# Autodesk Inventor assembly: Intake
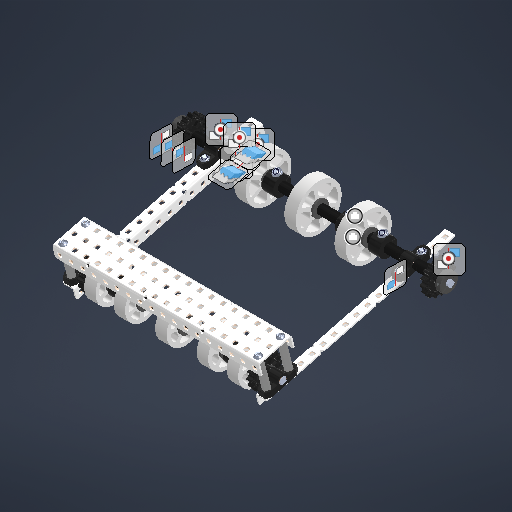
[picture p0: Inventor's stored thumbnail of the model, 512x512]
Saved by Autodesk Inventor 2025 (Build 290162000, 162)
## iProperties
Created: 2024-12-18
Part Number: Intake
Document SubType Name: Assembly
Designer: Juan
Author: Juan
## Documents named in this file (26)
- C:\Users\Juan\Documents\GitHub\ATUM-VRC-High-Stakes-CAD\Protobot\Intake.iam
- C:\Users\Juan\Documents\GitHub\ATUM-VRC-High-Stakes-CAD\VEX-CAD-Inventor\Motion\Shaft HS\Shaft HS\Shaft HS 9.0 in.ipt
- C:\Users\Juan\Documents\GitHub\ATUM-VRC-High-Stakes-CAD\VEX-CAD-Inventor\Motion\Shaft HS\Shaft HS.ipt
- C:\Users\Juan\Documents\GitHub\ATUM-VRC-High-Stakes-CAD\VEX-CAD-Inventor\Structure\Angle\Aluminum 1x1\Alu Angle 1x1x17.ipt
- C:\Users\Juan\Documents\GitHub\ATUM-VRC-High-Stakes-CAD\VEX-CAD-Inventor\Motion\Shaft HS\HS Pillow Bearing Block.ipt
- C:\Users\Juan\Documents\GitHub\ATUM-VRC-High-Stakes-CAD\VEX-CAD-Inventor\Motion\Sprockets\6P Sprocket\6P 16T Sprocket, No Insert.iam
- C:\Users\Juan\Documents\GitHub\ATUM-VRC-High-Stakes-CAD\VEX-CAD-Inventor\Motion\Sprockets\6P Sprocket.iam
- C:\Users\Juan\Documents\GitHub\ATUM-VRC-High-Stakes-CAD\VEX-CAD-Inventor\Structure\Hardware\Screw Steel - Star\SScrew Star Threaded .375.ipt
- C:\Users\Juan\Documents\GitHub\ATUM-VRC-High-Stakes-CAD\VEX-CAD-Inventor\Structure\Hardware\Screw Steel - Star.ipt
- C:\Users\Juan\Documents\GitHub\ATUM-VRC-High-Stakes-CAD\VEX-CAD-Inventor\Structure\C Channel\Aluminum 1x3x1\Alu C 1x3x1x18.ipt
- C:\Users\Juan\Documents\GitHub\ATUM-VRC-High-Stakes-CAD\VEX-CAD-Inventor\Structure\Standoff\Standoff 1.50.ipt
- C:\Users\Juan\Documents\GitHub\ATUM-VRC-High-Stakes-CAD\VEX-CAD-Inventor\Structure\Standoff.ipt
- C:\Users\Juan\Documents\GitHub\ATUM-VRC-High-Stakes-CAD\VEX-CAD-Inventor\Motion\1-Post Bearing Flat Hex Retainer.ipt
- C:\Users\Juan\Documents\GitHub\ATUM-VRC-High-Stakes-CAD\VEX-CAD-Inventor\Motion\Shaft HS\Shaft HS\Shaft HS 12.0 in.ipt
- C:\Users\Juan\Documents\GitHub\ATUM-VRC-High-Stakes-CAD\VEX-CAD-Inventor\Motion\Shaft HS\HS Shaft Collar.ipt
- C:\Users\Juan\Documents\GitHub\ATUM-VRC-High-Stakes-CAD\VEX-CAD-Inventor\Motion\Shaft HS\HS Spacer\HSpacer .5000.ipt
- C:\Users\Juan\Documents\GitHub\ATUM-VRC-High-Stakes-CAD\VEX-CAD-Inventor\Motion\Shaft HS\HS Spacer.ipt
- C:\Users\Juan\Documents\GitHub\ATUM-VRC-High-Stakes-CAD\VEX-CAD-Inventor\Motion\Shaft HS\Low Profile HS Shaft Collar.ipt
- C:\Users\Juan\Documents\GitHub\ATUM-VRC-High-Stakes-CAD\VEX-CAD-Inventor\Motion\Shaft HS\HS Spacer\HSpacer .2500.ipt
- C:\Users\Juan\Documents\GitHub\ATUM-VRC-High-Stakes-CAD\Protobot\2.0 Flex Wheel with Insert.iam
- C:\Users\Juan\Documents\GitHub\ATUM-VRC-High-Stakes-CAD\VEX-CAD-Inventor\Structure\Hardware\Nut Thin Nylock.ipt
- C:\Users\Juan\Documents\GitHub\ATUM-VRC-High-Stakes-CAD\VEX-CAD-Inventor\Structure\Hardware\Screw Steel - Star\SScrew Star Smooth .625.ipt
- C:\Users\Juan\Documents\GitHub\ATUM-VRC-High-Stakes-CAD\VEX-CAD-Inventor\Motion\Shaft HS\HS Spacer\HSpacer .1250.ipt
- C:\Users\Juan\Documents\GitHub\ATUM-VRC-High-Stakes-CAD\VEX-CAD-Inventor\Motion\Shaft HS\HS Spacer\HSpacer .0625.ipt
- C:\Users\Juan\Documents\GitHub\ATUM-VRC-High-Stakes-CAD\VEX-CAD-Inventor\Structure\Hardware\Screw Steel - Star\SScrew Star Smooth .375.ipt
- C:\Users\Juan\Documents\GitHub\ATUM-VRC-High-Stakes-CAD\Protobot\1.625 Flex Wheel with Insert.iam
## Components (88 placed, 20 different names)
1. Shaft HS 9.0 in:1
2. Alu Angle 1x1x17:1
3. HS Pillow Bearing Block:4
4. Alu Angle 1x1x17:2
5. HS Pillow Bearing Block:1
6. HS Pillow Bearing Block:2
7. 6P 16T Sprocket, No Insert:1 [sub-assembly]
8. 6P 16T Sprocket, No Insert:2 [sub-assembly]
9. SScrew Star Threaded .375:1
10. Alu C 1x3x1x18:1
11. Standoff 1.50:1
12. Standoff 1.50:2
13. Standoff 1.50:3
14. Standoff 1.50:4
15. 1-Post Bearing Flat Hex Retainer:1
16. HS Pillow Bearing Block:3
17. Shaft HS 12.0 in:2
18. 6P 16T Sprocket, No Insert:3 [sub-assembly]
19. 6P 16T Sprocket, No Insert:4 [sub-assembly]
20. HS Shaft Collar:1
21. HS Shaft Collar:2
22. HSpacer .5000:1
23. HSpacer .5000:2
24. HSpacer .5000:3
25. HSpacer .5000:4
26. Low Profile HS Shaft Collar:1
27. Low Profile HS Shaft Collar:2
28. HS Shaft Collar:3
29. HS Shaft Collar:4
30. HSpacer .2500:5
31. HSpacer .2500:6
32. 2.0 Flex Wheel with Insert:1 [sub-assembly]
33. 2.0 Flex Wheel with Insert:2 [sub-assembly]
34. 2.0 Flex Wheel with Insert:3 [sub-assembly]
35. HSpacer .5000:7
36. Nut Thin Nylock:1
37. HSpacer .5000:8
38. SScrew Star Smooth .625:2
39. SScrew Star Smooth .625:3
40. SScrew Star Smooth .625:4
41. SScrew Star Smooth .625:5
42. Nut Thin Nylock:2
43. Nut Thin Nylock:3
44. Nut Thin Nylock:4
45. HSpacer .5000:9
46. HSpacer .5000:10
47. HSpacer .1250:11
48. HSpacer .1250:12
49. HSpacer .0625:13
50. HSpacer .1250:14
51. HSpacer .1250:15
52. HSpacer .0625:16
53. HSpacer .0625:17
54. Nut Thin Nylock:5
55. Nut Thin Nylock:6
56. Nut Thin Nylock:7
57. Nut Thin Nylock:8
58. SScrew Star Smooth .375:6
59. SScrew Star Smooth .375:7
60. SScrew Star Smooth .375:8
61. SScrew Star Smooth .375:9
62. SScrew Star Smooth .375:10
63. SScrew Star Smooth .375:11
64. SScrew Star Smooth .375:12
65. SScrew Star Smooth .375:13
66. SScrew Star Smooth .375:14
67. SScrew Star Smooth .375:15
68. SScrew Star Smooth .375:16
69. SScrew Star Smooth .375:17
70. 1.625 Flex Wheel with Insert:1 [sub-assembly]
71. 1.625 Flex Wheel with Insert:2 [sub-assembly]
72. 1.625 Flex Wheel with Insert:3 [sub-assembly]
73. 1.625 Flex Wheel with Insert:4 [sub-assembly]
74. 1.625 Flex Wheel with Insert:5 [sub-assembly]
75. HSpacer .5000:18
76. HSpacer .1250:19
77. HSpacer .1250:20
78. HSpacer .5000:21
79. HSpacer .5000:22
80. HSpacer .5000:23
81. HS Shaft Collar:5
82. Nut Thin Nylock:9
83. SScrew Star Smooth .625:18
84. HS Shaft Collar:6
85. Nut Thin Nylock:10
86. SScrew Star Smooth .625:19
87. HSpacer .1250:24
88. HSpacer .1250:25
## Relationships (158: Mate 117, WeldJoint 30, CylindricalJoint 9, Flush 1, Angle 1)
- [Mate]: Alu Angle 1x1x17:1 ↔ HS Pillow Bearing Block:1
- [Mate]: Alu Angle 1x1x17:1 ↔ HS Pillow Bearing Block:1
- [Mate]: Alu Angle 1x1x17:1 ↔ HS Pillow Bearing Block:1
- [Mate]: Shaft HS 9.0 in:1 ↔ HS Pillow Bearing Block:1
- [Mate]: Alu Angle 1x1x17:2 ↔ HS Pillow Bearing Block:2
- [Mate]: Alu Angle 1x1x17:2 ↔ HS Pillow Bearing Block:2
- [Mate]: Alu Angle 1x1x17:2 ↔ HS Pillow Bearing Block:2
- [Mate]: Shaft HS 9.0 in:1 ↔ HS Pillow Bearing Block:2
- [Mate]: Shaft HS 9.0 in:1 ↔ 6P 16T Sprocket, No Insert:2
- [Mate]: Shaft HS 9.0 in:1 ↔ 6P 16T Sprocket, No Insert:1
- [Mate]: Alu Angle 1x1x17:1 ↔ SScrew Star Threaded .375:1
- [Mate]: Alu Angle 1x1x17:1 ↔ 6P 16T Sprocket, No Insert:2
- [Mate]: Alu Angle 1x1x17:1 ↔ SScrew Star Threaded .375:1
- [Mate]: Alu Angle 1x1x17:1 ↔ Alu Angle 1x1x17:2
- [Mate]: HS Pillow Bearing Block:1 ↔ Standoff 1.50:1
- [Mate]: HS Pillow Bearing Block:1 ↔ Standoff 1.50:2
- [Mate]: HS Pillow Bearing Block:1 ↔ Standoff 1.50:1
- [Mate]: HS Pillow Bearing Block:1 ↔ Standoff 1.50:2
- [Mate]: Alu C 1x3x1x18:1 ↔ Standoff 1.50:1
- [Mate]: Alu C 1x3x1x18:1 ↔ Standoff 1.50:2
- [Mate]: Alu C 1x3x1x18:1 ↔ Standoff 1.50:2
- [Mate]: HS Pillow Bearing Block:2 ↔ Standoff 1.50:4
- [Mate]: HS Pillow Bearing Block:2 ↔ Standoff 1.50:3
- [Mate]: HS Pillow Bearing Block:2 ↔ Standoff 1.50:4
- [Mate]: HS Pillow Bearing Block:2 ↔ Standoff 1.50:3
- [Mate]: Alu C 1x3x1x18:1 ↔ Standoff 1.50:3
- [Mate]: Alu Angle 1x1x17:2 ↔ HS Pillow Bearing Block:3
- [Mate]: Alu Angle 1x1x17:2 ↔ HS Pillow Bearing Block:3
- [Mate]: Alu Angle 1x1x17:2 ↔ HS Pillow Bearing Block:3
- [Mate]: Shaft HS 12.0 in:2 ↔ 6P 16T Sprocket, No Insert:3
- [Mate]: Shaft HS 12.0 in:2 ↔ 6P 16T Sprocket, No Insert:4
- [Mate]: Shaft HS 12.0 in:2 ↔ 2.0 Flex Wheel with Insert:3
- [Mate]: Shaft HS 12.0 in:2 ↔ 2.0 Flex Wheel with Insert:2
- [Mate]: Shaft HS 12.0 in:2 ↔ 2.0 Flex Wheel with Insert:1
- [Mate]: Shaft HS 12.0 in:2 ↔ HSpacer .5000:4
- [Mate]: Shaft HS 12.0 in:2 ↔ HSpacer .5000:4
- [Mate]: Shaft HS 12.0 in:2 ↔ HS Shaft Collar:1
- [Mate]: Shaft HS 12.0 in:2 ↔ HS Shaft Collar:1
- [Mate]: Shaft HS 12.0 in:2 ↔ HSpacer .5000:1
- [Mate]: Shaft HS 12.0 in:2 ↔ HSpacer .5000:1
- [Mate]: HSpacer .5000:1 ↔ HSpacer .5000:4
- [Mate]: HS Shaft Collar:1 ↔ HSpacer .5000:4
- [Mate]: HS Shaft Collar:1 ↔ 2.0 Flex Wheel with Insert:3
- [Mate]: HSpacer .5000:1 ↔ 2.0 Flex Wheel with Insert:2
- [Mate]: Shaft HS 12.0 in:2 ↔ HS Shaft Collar:2
- [Mate]: Shaft HS 12.0 in:2 ↔ HS Shaft Collar:2
- [Mate]: Shaft HS 12.0 in:2 ↔ HSpacer .5000:3
- [Mate]: Shaft HS 12.0 in:2 ↔ HSpacer .5000:3
- [Mate]: Shaft HS 12.0 in:2 ↔ HSpacer .5000:2
- [Mate]: Shaft HS 12.0 in:2 ↔ HSpacer .5000:2
- [Mate]: HSpacer .5000:2 ↔ 2.0 Flex Wheel with Insert:2
- [Mate]: HSpacer .5000:2 ↔ HSpacer .5000:3
- [Mate]: HS Shaft Collar:2 ↔ HSpacer .5000:3
- [Mate]: HS Shaft Collar:2 ↔ 2.0 Flex Wheel with Insert:1
- [Mate] (36.1696 mm): Alu Angle 1x1x17:1 ↔ 2.0 Flex Wheel with Insert:3
- [Mate]: Shaft HS 12.0 in:2 ↔ Low Profile HS Shaft Collar:2
- [Mate]: Shaft HS 12.0 in:2 ↔ Low Profile HS Shaft Collar:2
- [Mate]: 6P 16T Sprocket, No Insert:3 ↔ Low Profile HS Shaft Collar:2
- [Mate]: Shaft HS 12.0 in:2 ↔ Low Profile HS Shaft Collar:1
- [Mate]: Shaft HS 12.0 in:2 ↔ Low Profile HS Shaft Collar:1
- [Mate]: 6P 16T Sprocket, No Insert:4 ↔ Low Profile HS Shaft Collar:1
- [Mate]: Shaft HS 12.0 in:2 ↔ HS Shaft Collar:3
- [Mate]: Shaft HS 12.0 in:2 ↔ HS Shaft Collar:3
- [Mate]: Shaft HS 12.0 in:2 ↔ HS Shaft Collar:4
- [Mate]: Shaft HS 12.0 in:2 ↔ HS Shaft Collar:4
- [Mate]: Shaft HS 12.0 in:2 ↔ HSpacer .2500:5
- [Mate]: Shaft HS 12.0 in:2 ↔ HSpacer .2500:5
- [Mate]: Shaft HS 12.0 in:2 ↔ HSpacer .2500:6
- [Mate]: Shaft HS 12.0 in:2 ↔ HSpacer .2500:6
- [Mate]: HSpacer .2500:6 ↔ 2.0 Flex Wheel with Insert:3
- [Mate]: HSpacer .2500:5 ↔ 2.0 Flex Wheel with Insert:1
- [Mate]: HS Shaft Collar:4 ↔ HSpacer .2500:5
- [Mate]: HS Shaft Collar:3 ↔ HSpacer .2500:6
- [WeldJoint]: HS Shaft Collar:3 ↔ SScrew Star Smooth .625:2
- [WeldJoint]: HS Shaft Collar:1 ↔ SScrew Star Smooth .625:5
- [WeldJoint]: HS Shaft Collar:2 ↔ SScrew Star Smooth .625:4
- [WeldJoint]: HS Shaft Collar:4 ↔ SScrew Star Smooth .625:3
- [WeldJoint]: HS Shaft Collar:3 ↔ Nut Thin Nylock:1
- [WeldJoint]: HS Shaft Collar:4 ↔ Nut Thin Nylock:2
- [WeldJoint]: HS Shaft Collar:2 ↔ Nut Thin Nylock:3
- [WeldJoint]: HS Shaft Collar:1 ↔ Nut Thin Nylock:4
- [WeldJoint]: HS Shaft Collar:3 ↔ HSpacer .5000:7
- [WeldJoint]: HS Shaft Collar:4 ↔ HSpacer .5000:9
- [Mate]: Shaft HS 12.0 in:2 ↔ HSpacer .5000:8
- [Mate]: 6P 16T Sprocket, No Insert:3 ↔ HSpacer .5000:8
- [Mate]: Shaft HS 12.0 in:2 ↔ HSpacer .5000:10
- [Mate]: 6P 16T Sprocket, No Insert:4 ↔ HSpacer .5000:10
- [Mate]: Shaft HS 12.0 in:2 ↔ HSpacer .1250:12
- [Mate]: HSpacer .5000:10 ↔ HSpacer .1250:12
- [Mate]: HSpacer .5000:9 ↔ HSpacer .1250:11
- [Mate]: HSpacer .5000:9 ↔ HSpacer .1250:11
- [Mate]: HSpacer .1250:11 ↔ HSpacer .0625:13
- [Mate]: HSpacer .1250:11 ↔ HSpacer .0625:13
- [Mate]: HSpacer .5000:8 ↔ HSpacer .1250:14
- [Mate]: HSpacer .5000:8 ↔ HSpacer .1250:14
- [Mate]: HSpacer .1250:14 ↔ HSpacer .0625:16
- [Mate]: HSpacer .1250:14 ↔ HSpacer .0625:16
- [Mate]: HSpacer .5000:7 ↔ HSpacer .1250:15
- [Mate]: HSpacer .5000:7 ↔ HSpacer .1250:15
- [Mate]: HSpacer .1250:15 ↔ HSpacer .0625:17
- [Mate]: HSpacer .1250:15 ↔ HSpacer .0625:17
- [WeldJoint]: HS Pillow Bearing Block:3 ↔ Nut Thin Nylock:7
- [WeldJoint]: HS Pillow Bearing Block:3 ↔ Nut Thin Nylock:8
- [WeldJoint]: Alu Angle 1x1x17:1 ↔ SScrew Star Smooth .375:6
- [WeldJoint]: Alu Angle 1x1x17:1 ↔ SScrew Star Smooth .375:7
- [WeldJoint]: Alu Angle 1x1x17:2 ↔ SScrew Star Smooth .375:9
- [WeldJoint]: Alu Angle 1x1x17:2 ↔ SScrew Star Smooth .375:8
- [WeldJoint]: Alu C 1x3x1x18:1 ↔ SScrew Star Smooth .375:11
- [WeldJoint]: Alu C 1x3x1x18:1 ↔ SScrew Star Smooth .375:10
- [WeldJoint]: Alu C 1x3x1x18:1 ↔ SScrew Star Smooth .375:12
- [WeldJoint]: Alu C 1x3x1x18:1 ↔ SScrew Star Smooth .375:13
- [WeldJoint]: Alu Angle 1x1x17:2 ↔ SScrew Star Smooth .375:15
- [WeldJoint]: Alu Angle 1x1x17:2 ↔ SScrew Star Smooth .375:14
- [WeldJoint]: Alu Angle 1x1x17:1 ↔ SScrew Star Smooth .375:17
- [WeldJoint]: Alu Angle 1x1x17:1 ↔ SScrew Star Smooth .375:16
- [CylindricalJoint]: Shaft HS 9.0 in:1 ↔ 1.625 Flex Wheel with Insert:1
- [CylindricalJoint]: Shaft HS 9.0 in:1 ↔ 1.625 Flex Wheel with Insert:5
- [Mate]: 1.625 Flex Wheel with Insert:5 ↔ HSpacer .5000:18
- [Mate]: 1.625 Flex Wheel with Insert:5 ↔ HSpacer .1250:19
- [Mate]: 1.625 Flex Wheel with Insert:5 ↔ HSpacer .1250:19
- [Mate]: HSpacer .5000:18 ↔ HSpacer .1250:19
- [Mate]: 1.625 Flex Wheel with Insert:5 ↔ HSpacer .1250:20
- [Mate]: 1.625 Flex Wheel with Insert:5 ↔ HSpacer .1250:20
- [Mate]: 1.625 Flex Wheel with Insert:5 ↔ HSpacer .5000:21
- [Mate]: HSpacer .1250:20 ↔ HSpacer .5000:21
- [Mate]: 1.625 Flex Wheel with Insert:5 ↔ HSpacer .5000:23
- [Mate]: HSpacer .5000:18 ↔ HSpacer .5000:23
- [Mate]: 1.625 Flex Wheel with Insert:5 ↔ HSpacer .5000:22
- [Mate]: HSpacer .5000:21 ↔ HSpacer .5000:22
- [Mate]: 1.625 Flex Wheel with Insert:1 ↔ HSpacer .5000:23
- [CylindricalJoint]: Shaft HS 9.0 in:1 ↔ 1.625 Flex Wheel with Insert:4
- [Mate]: 1.625 Flex Wheel with Insert:4 ↔ HSpacer .5000:22
- [CylindricalJoint]: Shaft HS 9.0 in:1 ↔ 1.625 Flex Wheel with Insert:3
- [CylindricalJoint]: Shaft HS 9.0 in:1 ↔ 1.625 Flex Wheel with Insert:2
- [WeldJoint]: HS Shaft Collar:5 ↔ SScrew Star Smooth .625:18
- [WeldJoint]: HS Shaft Collar:5 ↔ Nut Thin Nylock:9
- [WeldJoint]: HS Shaft Collar:6 ↔ SScrew Star Smooth .625:19
- [WeldJoint]: HS Shaft Collar:6 ↔ Nut Thin Nylock:10
- [CylindricalJoint]: Shaft HS 9.0 in:1 ↔ HS Shaft Collar:5
- [CylindricalJoint]: Shaft HS 9.0 in:1 ↔ HS Shaft Collar:6
- [Mate]: 6P 16T Sprocket, No Insert:1 ↔ 1.625 Flex Wheel with Insert:2
- [Mate]: 1.625 Flex Wheel with Insert:2 ↔ HS Shaft Collar:6
- [Mate]: 6P 16T Sprocket, No Insert:2 ↔ 1.625 Flex Wheel with Insert:3
- [Mate]: 1.625 Flex Wheel with Insert:3 ↔ HS Shaft Collar:5
- [Mate]: Alu Angle 1x1x17:2 ↔ 6P 16T Sprocket, No Insert:1
- [Flush]: HS Shaft Collar:5 ↔ HS Shaft Collar:6
- [Angle] (0 deg): Shaft HS 9.0 in:1 ↔ HS Shaft Collar:5
- [CylindricalJoint]: Shaft HS 9.0 in:1 ↔ HSpacer .1250:25
- [Mate]: HS Shaft Collar:5 ↔ HSpacer .1250:25
- [Mate]: 1.625 Flex Wheel with Insert:1 ↔ HSpacer .1250:25
- [CylindricalJoint]: Shaft HS 9.0 in:1 ↔ HSpacer .1250:24
- [Mate]: 1.625 Flex Wheel with Insert:4 ↔ HSpacer .1250:24
- [Mate]: Alu Angle 1x1x17:1 ↔ HS Pillow Bearing Block:4
- [Mate]: Alu Angle 1x1x17:1 ↔ HS Pillow Bearing Block:4
- [Mate]: Alu Angle 1x1x17:1 ↔ HS Pillow Bearing Block:4
- [Mate]: HS Pillow Bearing Block:4 ↔ Shaft HS 12.0 in:2
- [WeldJoint]: HS Pillow Bearing Block:4 ↔ Nut Thin Nylock:6
- [WeldJoint]: HS Pillow Bearing Block:4 ↔ Nut Thin Nylock:5
## Named parameters: d2183_d2114 = 0 mm, d2184_d2118 = 0 mm, d2185_d2183_d2114 = 0 mm, d2186_d2184_d2118 = 0 mm
